# Autodesk Inventor assembly: Door Assembly
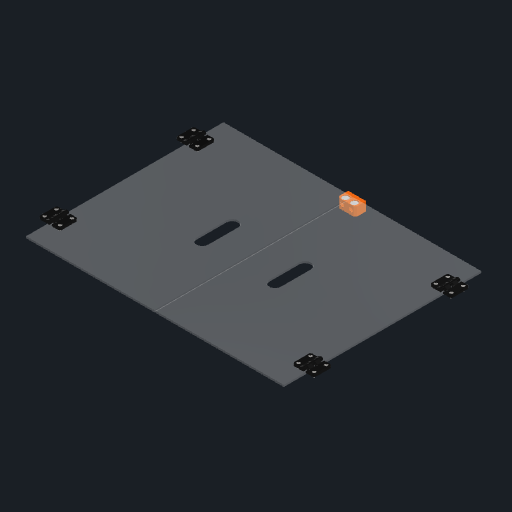
[picture p0: Inventor's stored thumbnail of the model, 512x512]
Saved by Autodesk Inventor 2023.1 (Build 271208000, 208)
## iProperties
Created: 2023-03-04
Part Number: Door Assembly
Document SubType Name: Assembly
Designer: remop
Author: remop
## Documents named in this file (6)
- C:\Users\remop\OneDrive\Documents\Inventor\3D Printers\LuEVO\Mk5_FullKinematic\Frame and Panels\Door\Door Assembly.iam
- C:\Users\remop\OneDrive\Documents\Inventor\3D Printers\LuEVO\Mk5_FullKinematic\Frame and Panels\Door\Door Base Magnet.ipt
- C:\Users\remop\OneDrive\Documents\Inventor\3D Printers\LuEVO\Mk4-Toolchanger\MagToolChanger_Magnet.ipt
- C:\Users\remop\OneDrive\Documents\Inventor\3D Printers\LuEVO\Mk5_FullKinematic\Frame and Panels\Door\Hinge_36x30_a270_4mm_printinplace.ipt
- C:\Users\remop\OneDrive\Documents\Inventor\3D Printers\LuEVO\Mk5_FullKinematic\Frame and Panels\Door\Door Panel.ipt
- C:\Users\remop\OneDrive\Documents\Inventor\Content Center Files\R2023\en-US\AS 1427(04)\AS 1427 - M3 x 8(5) I.ipt
## Components (24 placed, 5 different names)
1. Door Base Magnet:1 — Rigid:1, Rigid:2, Mate:1, Flush:8, Flush:9, Mate:2
2. MagToolChanger_Magnet:1 — Rigid:1
3. MagToolChanger_Magnet:2 — Rigid:2
4. Hinge_36x30_a270_4mm_printinplace:1 — Flush:3, Flush:4, Flush:5, Flush:6, Flush:8, Mate:3, Mate:4, Rigid:3, Rigid:4, Rigid:5, Rigid:6
5. Hinge_36x30_a270_4mm_printinplace:2 — Flush:1, Flush:2, Flush:5, Flush:6, Mate:1, Rigid:11, Rigid:12, Rigid:13, Rigid:14
6. Hinge_36x30_a270_4mm_printinplace:3 — Flush:1, Flush:2, Flush:7, Flush:9, Rigid:15, Rigid:16, Rigid:17, Rigid:18
7. Hinge_36x30_a270_4mm_printinplace:4 — Flush:3, Flush:4, Flush:7, Mate:2, Mate:3, Rigid:7, Rigid:8, Rigid:9, Rigid:10
8. Door Panel:1 — Mate:4
9. AS 1427 H - Metric M3 x 8:1 — Rigid:6
10. AS 1427 H - Metric M3 x 8:2 — Rigid:7
11. AS 1427 H - Metric M3 x 8:3 — Rigid:5
12. AS 1427 H - Metric M3 x 8:4 — Rigid:8
13. AS 1427 H - Metric M3 x 8:5 — Rigid:9
14. AS 1427 H - Metric M3 x 8:6 — Rigid:4
15. AS 1427 H - Metric M3 x 8:7 — Rigid:10
16. AS 1427 H - Metric M3 x 8:8 — Rigid:3
17. AS 1427 H - Metric M3 x 8:9 — Rigid:14
18. AS 1427 H - Metric M3 x 8:10 — Rigid:13
19. AS 1427 H - Metric M3 x 8:11 — Rigid:15
20. AS 1427 H - Metric M3 x 8:12 — Rigid:16
21. AS 1427 H - Metric M3 x 8:13 — Rigid:17
22. AS 1427 H - Metric M3 x 8:14 — Rigid:12
23. AS 1427 H - Metric M3 x 8:15 — Rigid:11
24. AS 1427 H - Metric M3 x 8:16 — Rigid:18
## Relationships (31: WeldJoint 18, Flush 9, Mate 4)
- Rigid:1 [WeldJoint]: Door Base Magnet:1 ↔ MagToolChanger_Magnet:1
- Rigid:2 [WeldJoint]: Door Base Magnet:1 ↔ MagToolChanger_Magnet:2
- Flush:1: Hinge_36x30_a270_4mm_printinplace:2 ↔ Hinge_36x30_a270_4mm_printinplace:3
- Flush:2: Hinge_36x30_a270_4mm_printinplace:2 ↔ Hinge_36x30_a270_4mm_printinplace:3
- Flush:3: Hinge_36x30_a270_4mm_printinplace:1 ↔ Hinge_36x30_a270_4mm_printinplace:4
- Flush:4: Hinge_36x30_a270_4mm_printinplace:1 ↔ Hinge_36x30_a270_4mm_printinplace:4
- Flush:5: Hinge_36x30_a270_4mm_printinplace:1 ↔ Hinge_36x30_a270_4mm_printinplace:2
- Flush:6: Hinge_36x30_a270_4mm_printinplace:1 ↔ Hinge_36x30_a270_4mm_printinplace:2
- Flush:7: Hinge_36x30_a270_4mm_printinplace:3 ↔ Hinge_36x30_a270_4mm_printinplace:4
- Mate:1 (3 mm): Door Base Magnet:1 ↔ Hinge_36x30_a270_4mm_printinplace:2
- Flush:8 (210 mm): Door Base Magnet:1 ↔ Hinge_36x30_a270_4mm_printinplace:1
- Flush:9 (210 mm): Door Base Magnet:1 ↔ Hinge_36x30_a270_4mm_printinplace:3
- Mate:2 (25 mm): Door Base Magnet:1 ↔ Hinge_36x30_a270_4mm_printinplace:4
- Mate:3 (200 mm): Hinge_36x30_a270_4mm_printinplace:1 ↔ Hinge_36x30_a270_4mm_printinplace:4
- Mate:4: Hinge_36x30_a270_4mm_printinplace:1 ↔ Door Panel:1
- Rigid:3 [WeldJoint]: Hinge_36x30_a270_4mm_printinplace:1 ↔ AS 1427 H - Metric M3 x 8:8
- Rigid:4 [WeldJoint]: Hinge_36x30_a270_4mm_printinplace:1 ↔ AS 1427 H - Metric M3 x 8:6
- Rigid:5 [WeldJoint]: Hinge_36x30_a270_4mm_printinplace:1 ↔ AS 1427 H - Metric M3 x 8:3
- Rigid:6 [WeldJoint]: Hinge_36x30_a270_4mm_printinplace:1 ↔ AS 1427 H - Metric M3 x 8:1
- Rigid:7 [WeldJoint]: Hinge_36x30_a270_4mm_printinplace:4 ↔ AS 1427 H - Metric M3 x 8:2
- Rigid:8 [WeldJoint]: Hinge_36x30_a270_4mm_printinplace:4 ↔ AS 1427 H - Metric M3 x 8:4
- Rigid:9 [WeldJoint]: Hinge_36x30_a270_4mm_printinplace:4 ↔ AS 1427 H - Metric M3 x 8:5
- Rigid:10 [WeldJoint]: Hinge_36x30_a270_4mm_printinplace:4 ↔ AS 1427 H - Metric M3 x 8:7
- Rigid:11 [WeldJoint]: Hinge_36x30_a270_4mm_printinplace:2 ↔ AS 1427 H - Metric M3 x 8:15
- Rigid:12 [WeldJoint]: Hinge_36x30_a270_4mm_printinplace:2 ↔ AS 1427 H - Metric M3 x 8:14
- Rigid:13 [WeldJoint]: Hinge_36x30_a270_4mm_printinplace:2 ↔ AS 1427 H - Metric M3 x 8:10
- Rigid:14 [WeldJoint]: Hinge_36x30_a270_4mm_printinplace:2 ↔ AS 1427 H - Metric M3 x 8:9
- Rigid:15 [WeldJoint]: Hinge_36x30_a270_4mm_printinplace:3 ↔ AS 1427 H - Metric M3 x 8:11
- Rigid:16 [WeldJoint]: Hinge_36x30_a270_4mm_printinplace:3 ↔ AS 1427 H - Metric M3 x 8:12
- Rigid:17 [WeldJoint]: Hinge_36x30_a270_4mm_printinplace:3 ↔ AS 1427 H - Metric M3 x 8:13
- Rigid:18 [WeldJoint]: Hinge_36x30_a270_4mm_printinplace:3 ↔ AS 1427 H - Metric M3 x 8:16
